# Autodesk Inventor assembly: Assembly2
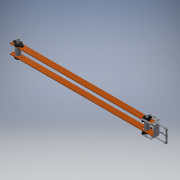
[picture p0: Inventor's stored thumbnail of the model, 180x180]
Saved by Autodesk Inventor 2019 (Build 230136000, 136)
## iProperties
Created: 2021-11-02
Part Number: Assembly2
Document SubType Name: Assembly
Designer: modym
Author: modym
## iProperties of the stored document bearing.ipt
Created: 2021-11-02
Part Number: bearing
Material: Generic
Document SubType Name: Modeling
Designer: modym
Density: 1 g/cm^3
Appearance: Default
Author: modym
## iProperties of the stored document tobolttoconnectorscccccc.ipt
Created: 2021-11-02
Part Number: tobolttoconnectorscccccc
Material: Generic
Document SubType Name: Modeling
Designer: modym
Density: 1 g/cm^3
Appearance: Default
Author: modym
## iProperties of the stored document rodddz.iam
Created: 2021-11-02
Part Number: rodddz
Document SubType Name: Assembly
Designer: modym
Sending System: Autodesk Inventor 2019
Preprocessor: ST-DEVELOPER v17
Title: C:\Users\modym\OneDrive\Desktop\Final version\rodddz.stp
Author: modym
## iProperties of the stored document tension_connector_rod1.ipt
Created: 2021-11-02
Part Number: tension_connector_rod1
Material: Generic
Document SubType Name: Modeling
Designer: modym
Density: 1 g/cm^3
Appearance: Default
Author: modym
## iProperties of the stored document rodddz.iam
Created: 2021-11-02
Part Number: rodddz
Document SubType Name: Assembly
Designer: modym
Author: modym
## iProperties of the stored document t.ipt
Created: 2021-11-02
Part Number: t
Material: Generic
Document SubType Name: Modeling
Designer: modym
Density: 1 g/cm^3
Appearance: Default
Author: modym
## iProperties of the stored document ccccccc.ipt
Created: 2021-11-02
Part Number: ccccccc
Material: Generic
Document SubType Name: Modeling
Designer: modym
Density: 1 g/cm^3
Appearance: Default
Author: modym
## iProperties of the stored document tension_connector.ipt
Created: 2021-11-02
Part Number: tension_connector
Material: Generic
Document SubType Name: Modeling
Designer: modym
Density: 1 g/cm^3
Appearance: Default
Author: modym
## Documents named in this file (18)
- **C:\Users\modym\OneDrive\Desktop\Final version\Assembly2.iam*LocalDocs*xMfpcdummWy25eh0kVm2fbjnmEh*bearing.ipt
- **C:\Users\modym\OneDrive\Desktop\Final version\Assembly2.iam*LocalDocs*x4aq210m5HqyxujcdEt2qtm3bOh*tobolttoconnectorscccccc.ipt
- **C:\Users\modym\OneDrive\Desktop\Final version\Assembly2.iam*LocalDocs*x3fw1l2fw1jbau0k0Sjglvlhh1h*rodddz.iam
- **C:\Users\modym\OneDrive\Desktop\Final version\Assembly2.iam*LocalDocs*xSv1yd1jbW2lcexwzBnr5ueyxWg*rodddz.iam
- **C:\Users\modym\OneDrive\Desktop\Final version\Assembly2.iam*LocalDocs*xTdyzpbggFtqwedgjDqe4wkcyFc*ccccccc.ipt
- **C:\Users\modym\OneDrive\Desktop\Final version\Assembly2.iam*LocalDocs*xRrajnp2wNrtpuvgeBkfrszqsTa*t.ipt
- **C:\Users\modym\OneDrive\Desktop\Final version\Assembly2.iam*LocalDocs*xJzqu1ai4Arlhek4eWmhibnhsPa*tension_connector_rod1.ipt
- **C:\Users\modym\OneDrive\Desktop\Final version\Assembly2.iam*LocalDocs*xTmpzw2kyUomkuu01Rc2p4zqz5b*tension_connector.ipt
- C:\Users\modym\OneDrive\Desktop\Final version\Assembly2.iam
- C:\Users\modym\OneDrive\Desktop\Final version\convyerwall.ipt
- C:\Users\modym\OneDrive\Desktop\Final version\convyerwall2.ipt
- C:\Users\modym\OneDrive\Desktop\Final version\flange.ipt
- C:\Users\modym\OneDrive\Desktop\Final version\rolling.ipt
- C:\Users\modym\OneDrive\Desktop\Final version\bolt.ipt
- C:\Users\modym\OneDrive\Desktop\Final version\nut.ipt
- C:\Users\modym\OneDrive\Desktop\Final version\bearing.ipt
- C:\Users\modym\OneDrive\Desktop\Final version\coupler.ipt
- C:\Users\modym\OneDrive\Desktop\Final version\rodddz.stp
## Components (11 placed, 9 different names)
1. convyerwall:1 — Mate:2, Mate:3, Mate:5, Mate:9, Mate:10, Mate:11, Mate:22
2. convyerwall2:1 — Mate:1, Mate:4, Mate:6, Mate:7, Mate:8, Flush:1, Mate:21, Mate:24
3. flange:1 — Mate:6, Mate:7, Flush:1, Mate:13, Mate:18
4. rolling:1 — Mate:1, Mate:2, Mate:3, Mate:4, Mate:19, Mate:20, Mate:25, Mate:26
5. rolling:2 — Mate:5, Mate:8, Mate:9, Mate:10, Mate:12
6. rodddz:1 [sub-assembly] — Mate:11, Mate:12, Mate:16, Mate:17
7. bolt:1 — Mate:15, Mate:16, Mate:17
8. nut:1 — Mate:13, Mate:15, Mate:18
9. bearing:1 — Mate:19, Mate:22, Mate:23
10. bearing:2 — Mate:20, Mate:21, Mate:23, Mate:24
11. coupler:1 — Mate:25, Mate:26
## Relationships (26: Mate 25, Flush 1)
- Mate:1: convyerwall2:1 ↔ rolling:1
- Mate:2: convyerwall:1 ↔ rolling:1
- Mate:3 (5 mm): convyerwall:1 ↔ rolling:1
- Mate:4 (5 mm): convyerwall2:1 ↔ rolling:1
- Mate:5 (5 mm): convyerwall:1 ↔ rolling:2
- Mate:6: convyerwall2:1 ↔ flange:1
- Mate:7: convyerwall2:1 ↔ flange:1
- Mate:8 (10.5 mm): convyerwall2:1 ↔ rolling:2
- Mate:9 (10.5 mm): convyerwall:1 ↔ rolling:2
- Mate:10 (10.2 mm): convyerwall:1 ↔ rolling:2
- Flush:1: convyerwall2:1 ↔ flange:1
- Mate:11: convyerwall:1 ↔ rodddz:1
- Mate:12: rolling:2 ↔ rodddz:1
- Mate:13: flange:1 ↔ nut:1
- Mate:15: bolt:1 ↔ nut:1
- Mate:16: rodddz:1 ↔ bolt:1
- Mate:17: rodddz:1 ↔ bolt:1
- Mate:18: flange:1 ↔ nut:1
- Mate:19: rolling:1 ↔ bearing:1
- Mate:20: rolling:1 ↔ bearing:2
- Mate:21: convyerwall2:1 ↔ bearing:2
- Mate:22: convyerwall:1 ↔ bearing:1
- Mate:23: bearing:1 ↔ bearing:2
- Mate:24: convyerwall2:1 ↔ bearing:2
- Mate:25: rolling:1 ↔ coupler:1
- Mate:26 (2 mm): rolling:1 ↔ coupler:1
